# Autodesk Inventor assembly: Toggle_Switch
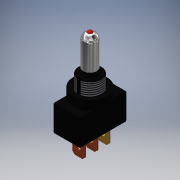
[picture p0: Inventor's stored thumbnail of the model, 180x180]
Saved by Autodesk Inventor 2016 (Build 200138000, 138)
## iProperties
Created: 2016-04-13
Part Number: Toggle_Switch
Document SubType Name: Assembly
Designer: agmle
Author: agmle
## Documents named in this file (8)
- C:\Users\agmle\BitTorrent Sync\private\projects\Creekfleet_Timer\hardware\CAD\Main\Toggle_Switch.iam
- C:\Users\agmle\BitTorrent Sync\private\projects\Creekfleet_Timer\hardware\CAD\Main\Toggle_Base.ipt
- C:\Users\agmle\BitTorrent Sync\private\projects\Creekfleet_Timer\hardware\CAD\Main\Toggle_Lever.ipt
- C:\Users\agmle\BitTorrent Sync\private\projects\Creekfleet_Timer\hardware\CAD\Main\Toggle_Cap.ipt
- C:\Users\agmle\BitTorrent Sync\private\projects\Creekfleet_Timer\hardware\CAD\Main\Toggle_LED.ipt
- C:\Users\agmle\BitTorrent Sync\private\projects\Creekfleet_Timer\hardware\CAD\Main\Toggle_Collar.ipt
- C:\Users\agmle\BitTorrent Sync\private\projects\Creekfleet_Timer\hardware\CAD\Main\Toggle_Pin_Brass.ipt
- C:\Users\agmle\BitTorrent Sync\private\projects\Creekfleet_Timer\hardware\CAD\Main\Toggle_Pin_Copper.ipt
## Components (8 placed, 7 different names)
1. Toggle_Base:1 — Mate:1, Mate:2, Mate:3, Mate:4, Angle:1, Mate:5, Mate:6, Angle:2, Mate:11, Flush:3, Flush:4
2. Toggle_Lever:1 — Mate:3, Mate:4, Angle:1, Insert:1
3. Toggle_Cap:1 — Insert:1, Insert:2
4. Toggle_LED:1 — Insert:2
5. Toggle_Collar:1 — Mate:5, Mate:6, Angle:2
6. Toggle_Pin_Brass:1 — Mate:8, Mate:9, Flush:1, Flush:3, Flush:4
7. Toggle_Pin_Copper:1 — Mate:7, Mate:10, Flush:2
8. Toggle_Pin_Copper:2 — Mate:7, Mate:8, Mate:9, Mate:10, Flush:1, Flush:2, Mate:11
## Relationships (19: Mate 11, Flush 4, Angle 2, Insert 2)
- Mate:1: Toggle_Base:1
- Mate:2: Toggle_Base:1
- Mate:3 (1.8 mm): Toggle_Base:1 ↔ Toggle_Lever:1
- Mate:4: Toggle_Base:1 ↔ Toggle_Lever:1
- Angle:1 (0 deg): Toggle_Base:1 ↔ Toggle_Lever:1
- Insert:1: Toggle_Lever:1 ↔ Toggle_Cap:1
- Insert:2 (-0.5 mm): Toggle_Cap:1 ↔ Toggle_LED:1
- Mate:5: Toggle_Base:1 ↔ Toggle_Collar:1
- Mate:6: Toggle_Base:1 ↔ Toggle_Collar:1
- Angle:2 (0 deg): Toggle_Base:1 ↔ Toggle_Collar:1
- Mate:7: Toggle_Pin_Copper:1 ↔ Toggle_Pin_Copper:2
- Mate:8: Toggle_Pin_Brass:1 ↔ Toggle_Pin_Copper:2
- Mate:9 (5.5 mm): Toggle_Pin_Brass:1 ↔ Toggle_Pin_Copper:2
- Mate:10 (5.7 mm): Toggle_Pin_Copper:1 ↔ Toggle_Pin_Copper:2
- Flush:1: Toggle_Pin_Brass:1 ↔ Toggle_Pin_Copper:2
- Flush:2: Toggle_Pin_Copper:1 ↔ Toggle_Pin_Copper:2
- Mate:11: Toggle_Base:1 ↔ Toggle_Pin_Copper:2
- Flush:3 (5 mm): Toggle_Base:1 ↔ Toggle_Pin_Brass:1
- Flush:4 (3.6 mm): Toggle_Base:1 ↔ Toggle_Pin_Brass:1
